# Autodesk Inventor assembly: Frez No,2
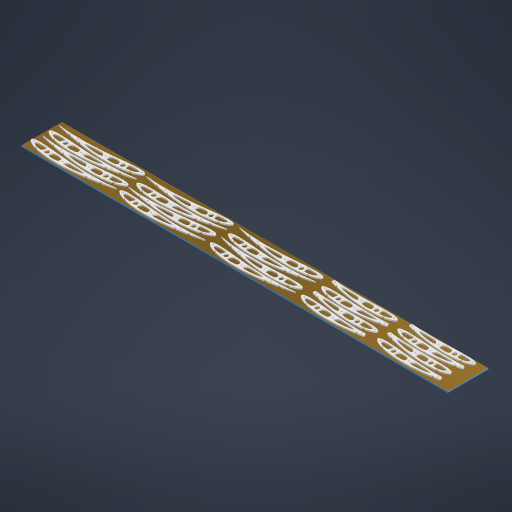
[picture p0: Inventor's stored thumbnail of the model, 512x512]
Saved by Autodesk Inventor 2023 (Build 270158000, 158)
## iProperties
Created: 2023-04-30
Part Number: Frez No,2
Document SubType Name: Assembly
Designer: szykr
Author: szykr
## Documents named in this file (4)
- D:\Folder Instalacyjny\GitHub Pliki\Solaris\new model\Frez_zebra\Frez No,2.iam
- D:\Folder Instalacyjny\GitHub Pliki\Solaris\new model\Frez_zebra\Balsa(95x1000x3).ipt
- D:\Folder Instalacyjny\GitHub Pliki\Solaris\new model\Żebro default.ipt
- D:\Folder Instalacyjny\GitHub Pliki\Solaris\new model\Żebro z lotką.ipt
## Components (21 placed, 3 different names)
1. Balsa(95x1000x3):1 — Mate:1, Mate:2, Mate:3, Mate:4, Mate:5, Mate:6, Mate:7, Mate:8, Mate:9, Mate:10, Mate:11, Mate:12, Mate:13, Mate:14, Mate:15, Mate:16, Mate:17, Mate:18, Mate:19, Mate:20
2. Żebro default:1 — Mate:4
3. Żebro default:2 — Mate:3
4. Żebro default:3 — Mate:2
5. Żebro default:4 — Mate:1
6. Żebro default:5 — Mate:7
7. Żebro default:6 — Mate:8
8. Żebro default:7 — Mate:6
9. Żebro default:8 — Mate:5
10. Żebro default:9 — Mate:11
11. Żebro default:10 — Mate:12
12. Żebro default:11 — Mate:10
13. Żebro default:12 — Mate:9
14. Żebro z lotką:1 — Mate:13
15. Żebro z lotką:2 — Mate:14
16. Żebro z lotką:3 — Mate:16
17. Żebro z lotką:4 — Mate:15
18. Żebro z lotką:5 — Mate:17
19. Żebro z lotką:6 — Mate:18
20. Żebro z lotką:7 — Mate:20
21. Żebro z lotką:8 — Mate:19
## Relationships (20: Mate 20)
- Mate:1: Balsa(95x1000x3):1 ↔ Żebro default:4
- Mate:2: Balsa(95x1000x3):1 ↔ Żebro default:3
- Mate:3: Balsa(95x1000x3):1 ↔ Żebro default:2
- Mate:4: Balsa(95x1000x3):1 ↔ Żebro default:1
- Mate:5: Balsa(95x1000x3):1 ↔ Żebro default:8
- Mate:6: Balsa(95x1000x3):1 ↔ Żebro default:7
- Mate:7: Balsa(95x1000x3):1 ↔ Żebro default:5
- Mate:8: Balsa(95x1000x3):1 ↔ Żebro default:6
- Mate:9: Balsa(95x1000x3):1 ↔ Żebro default:12
- Mate:10: Balsa(95x1000x3):1 ↔ Żebro default:11
- Mate:11: Balsa(95x1000x3):1 ↔ Żebro default:9
- Mate:12: Balsa(95x1000x3):1 ↔ Żebro default:10
- Mate:13: Balsa(95x1000x3):1 ↔ Żebro z lotką:1
- Mate:14: Balsa(95x1000x3):1 ↔ Żebro z lotką:2
- Mate:15: Balsa(95x1000x3):1 ↔ Żebro z lotką:4
- Mate:16: Balsa(95x1000x3):1 ↔ Żebro z lotką:3
- Mate:17: Balsa(95x1000x3):1 ↔ Żebro z lotką:5
- Mate:18: Balsa(95x1000x3):1 ↔ Żebro z lotką:6
- Mate:19: Balsa(95x1000x3):1 ↔ Żebro z lotką:8
- Mate:20: Balsa(95x1000x3):1 ↔ Żebro z lotką:7
